# Autodesk Inventor assembly: SCSW6-8
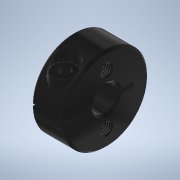
[picture p0: Inventor's stored thumbnail of the model, 180x180]
Saved by Autodesk Inventor 2022.3 (Build 263350000, 350)
## iProperties
Category: PARTsolutions
Company: MISUMI
Created: 2019-10-03
Part Number: SCSW6-8
Catalog Web Link: www.cadenas.de
Description: SCSW, PSCSW, SSCSW-Shaft Collars - 2-Tapped (Coarse Thread)
Vendor: MISUMI
Document SubType Name: Assembly
Designer: psadmin
Manufacturer: MISUMI
Mass: 2.06479 g
Surface Area: 17.3217 cm^2
Volume: 2.06479 cm^3
Density: 1 g/cm^3
PSOL_IDENT_0: {$CADENAS_DATA\23d-libs\misumi\metric\03_set_collars\scsw_asmtab.prj},192 {VTYP=3D},{STYP=ASSTAB},{N
PSOL_IDENT_1: B=SCSW6-8},{LINA=SCSW6-8},{NN=SCSW, PSCSW, SSCSW},{DATE=30.09.2019 14:56:54},{GEOMDATE=24.02.2016 04
PSOL_IDENT_2: :35:42},{VERSION=},{LINEID=220},{WBVAR=MAT,ST,BS},{WBNUMERIC=BS}  {NB=SCSW6-8},{LINA=SCSW6-8},{KT=DU
PSOL_IDENT_3: MMY},{PN=SCSW6-8},{TYPE=SCSW},{MAT=1045},{ST=Black Oxide},{AC=Hexagon Socket Head Set Screw 1 Pc.},{
PSOL_IDENT_4: D=6},{BS=8},{D1=20},{M=M3},{THMD=3},{THDMIN=2.459},{ST0='Black Oxide','Black Oxide','Electroless Nic
PSOL_IDENT_5: kel Plating','Electroless Nickel Plating'},{B1=8,10},{DD=3.4},{R=3.00},{W=1.0},{X=6.0},{Y=4.0},{Z=6~
PSOL_IDENT_6: 6.5},{S=3.5},{P=12},{C=0.5},{L=10},{M1=M3},{ZZ=6.25},{THMD1=3},{THDMIN1=2.459},{PPATH=scsw_templ.prj
PSOL_IDENT_7: }
NN: SCSW, PSCSW, SSCSW
NT: Shaft Collars - 2-Tapped (Coarse Thread)
NB: SCSW6-8
NBSYN: $PN.
LINA: SCSW6-8
PN: SCSW6-8
MAT: S45C Equivalent
ST: Black Oxide
AC: Hexagon Socket Head Set Screw 1 Pc.
D: 6
BS: 8
D1: 20
M: M3
DD: 3.4
R: 3
W: 1
X: 6
Y: 4
Z: 6~6.5
S: 3.5
P: 12
M1: M3
SUPPLIER: MISUMI
ARTICLENO: SCSW6-8
BOMINFO: SCSW6-8
CREATOR: CADENAS GmbH
Title: SCSW6-8
Author: Cadenas PARTsolutions
Comments: Shaft Collars - 2-Tapped (Coarse Thread)
## Documents named in this file (3)
- C:\Users\YusukeKunita\Documents\GrabCAD\Development\BasicParts\SetCollar\SCSW6-8\SCSW6-8.iam
- C:\Users\YusukeKunita\Documents\GrabCAD\Development\BasicParts\SetCollar\SCSW6-8\SCSW6-8b.ipt
- C:\Users\YusukeKunita\Documents\GrabCAD\Development\BasicParts\SetCollar\SCSW6-8\Slotted head cap screw ISO 4762 - M3x10.ipt
## Components (2 placed, 2 different names)
1. SCSW6-8b:1 — body_screw_Z@1 <-> IP1_Z@2
2. Slotted head cap screw ISO 4762 - M3x10:1 — body_screw_Z@1 <-> IP1_Z@2
## Relationships (1: Mate 1)
- body_screw_Z@1 <-> IP1_Z@2 [Mate]: SCSW6-8b:1 ↔ Slotted head cap screw ISO 4762 - M3x10:1
